# Autodesk Inventor assembly: Arm
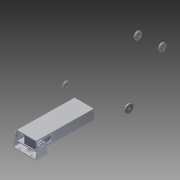
[picture p0: Inventor's stored thumbnail of the model, 180x180]
Saved by Autodesk Inventor 2013 (Build 170138000, 138)
## iProperties
Created: 2014-04-08
Part Number: Arm
Document SubType Name: Assembly
Designer: andou
Author: andou
## Documents named in this file (6)
- C:\Users\andou\Documents\GitHub\Robotics-Project\design\RoboticsProject\project_4\Arm.iam
- C:\Users\andou\Documents\GitHub\Robotics-Project\design\RoboticsProject\project_4\Generic Parts\KRS-2542HV.ipt
- C:\Users\andou\Documents\GitHub\Robotics-Project\design\RoboticsProject\project_4\Generic Parts\Low_Height_Horn.ipt
- C:\Users\andou\Documents\GitHub\Robotics-Project\design\RoboticsProject\project_4\Free_Horn.iam
- C:\Users\andou\Documents\GitHub\Robotics-Project\design\RoboticsProject\project_4\Bracket.ipt
- C:\Users\andou\Documents\GitHub\Robotics-Project\design\RoboticsProject\project_4\Arm_Link_Flame.ipt
## Components (9 placed, 5 different names)
1. KRS-2542HV:1 — 挿入:5, 挿入:6, 挿入:7
2. Low_Height_Horn:1 — 挿入:5, 挿入:9
3. Free_Horn:1 [sub-assembly]
4. Free_Horn:2 [sub-assembly]
5. Free_Horn:4 [sub-assembly] — 挿入:8, 挿入:10
6. Free_Horn:6 [sub-assembly]
7. Free_Horn:7 [sub-assembly]
8. Bracket:1 — 挿入:9, 挿入:10
9. Arm_Link_Flame:1 — 挿入:6, 挿入:7, 挿入:8
## Relationships (6: Insert 6)
- 挿入:5 [Insert]: KRS-2542HV:1 ↔ Low_Height_Horn:1
- 挿入:6 [Insert]: KRS-2542HV:1 ↔ Arm_Link_Flame:1
- 挿入:7 [Insert]: KRS-2542HV:1 ↔ Arm_Link_Flame:1
- 挿入:8 [Insert]: Free_Horn:4 ↔ Arm_Link_Flame:1
- 挿入:9 [Insert]: Low_Height_Horn:1 ↔ Bracket:1
- 挿入:10 [Insert]: Free_Horn:4 ↔ Bracket:1
